# Autodesk Inventor assembly: ASY GBK 1310 long wall shield 4
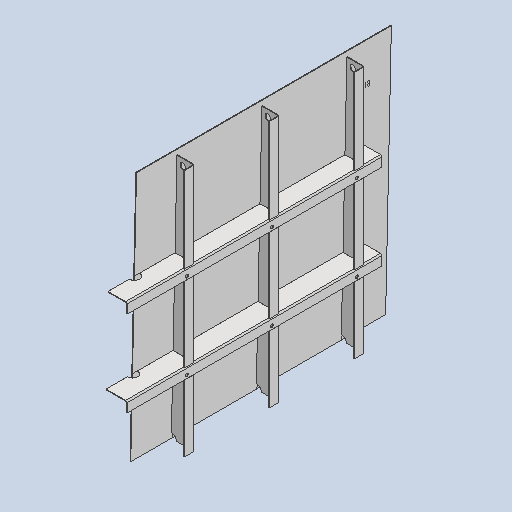
[picture p0: Inventor's stored thumbnail of the model, 512x512]
Saved by Autodesk Inventor 2026.3 (Build 303398000, 398)
## iProperties
Created: 2026-05-07
Part Number: ASY GBK 1310 long wall shield 4
Document SubType Name: Assembly
Designer: pokla
Mass: 107756 g
Surface Area: 69611.7 cm^2
Volume: 13726.9 cm^3
Stock Number: 1310
Author: admin
Comments: поменял
## Documents named in this file (6)
- C:\Users\admin\Documents\Inventor\GBK-Gubkinskiy\ASY GBK 1310 long wall shield 4.iam
- C:\Users\admin\Documents\Inventor\GBK-Gubkinskiy\GBK 1318 shield.ipt
- C:\Users\admin\Documents\Inventor\GBK-Gubkinskiy\GBK 0301 third rib.ipt
- C:\Users\admin\Documents\Inventor\GBK-Gubkinskiy\GBK 0302 stringer 7.ipt
- C:\Users\admin\Documents\Inventor\GBK-Gubkinskiy\GBK 0303 stringer 8.ipt
- C:\Users\admin\Documents\Inventor\GBK-Gubkinskiy\GBK 0101 main rib.ipt
## Components (6 placed, 4 different names)
1. GBK 0302 stringer 7:1
2. GBK 0303 stringer 8:1 — Flush:1
3. GBK 1318 shield:1 — Flush:1, Mate:3
4. GBK 0301 third rib:1 — Mate:4, Flush:2
5. GBK 0301 third rib:2
6. GBK 0301 third rib:3
## Component patterns: (3 elements, first: GBK 0301 third rib:1)
## Relationships (8: Mate 4, WeldJoint 2, Flush 2)
- [Mate]: GBK 1318 shield:1 ↔ GBK 0301 third rib:1
- [Mate]: GBK 1318 shield:1 ↔ GBK 0301 third rib:1
- [WeldJoint] (4 mm): GBK 0302 stringer 7:1 ↔ GBK 0301 third rib:1
- [WeldJoint] (4 mm): GBK 0303 stringer 8:1 ↔ GBK 0301 third rib:1
- Flush:1 (155 mm): GBK 0303 stringer 8:1 ↔ GBK 1318 shield:1
- Mate:3: GBK 1318 shield:1
- Mate:4: GBK 0301 third rib:1
- Flush:2: GBK 0301 third rib:1
## Named parameters: Шаг_шпангоутов = 496.66667 mm
